# Autodesk Inventor assembly: TEST ASEMBLY
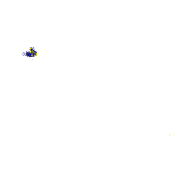
[picture p0: Inventor's stored thumbnail of the model, 180x180]
Saved by Autodesk Inventor 2019 (Build 230136000, 136)
## iProperties
Created: 2019-10-13
Part Number: TEST ASEMBLY
Document SubType Name: Assembly
Designer: Admin
Author: Admin
## Documents named in this file (21)
- C:\Users\Admin\Documents\TEST ASEMBLY.iam
- C:\Users\Admin\Documents\BASE FOR SYSTEM.ipt
- C:\Users\Admin\Documents\bolt for capping system.ipt
- C:\Users\Admin\Documents\bottom part of capping system.ipt
- C:\Users\Admin\Documents\nut for capping system.ipt
- C:\Users\Admin\Documents\without head nut for capping system.ipt
- C:\Users\Admin\Documents\cappingsystem 3rd part.ipt
- C:\Users\Admin\Documents\dc motor for capping system.ipt
- C:\Users\Admin\Documents\DC MOTOR NUT FOR CAPPING SYSTEM.ipt
- C:\Users\Admin\Documents\2 nd part of capping syStem.ipt
- C:\Users\Admin\Documents\two way connector for capping system.ipt
- C:\Users\Admin\Documents\CAPPER.ipt
- C:\Users\Admin\Documents\nut1.ipt
- C:\Users\Admin\Documents\STAND PLATE FOR STORSGE SYSTEM.ipt
- C:\Users\Admin\Documents\ir sensor.ipt
- C:\Users\Admin\Documents\top STAND PLATE FOR STORSGE SYSTEM.ipt
- C:\Users\Admin\Documents\Assembly3.iam
- C:\Users\Admin\Documents\ppe assembly.iam
- C:\Users\Admin\Documents\SA.ipt
- C:\Users\Admin\Documents\BOLT SMALL.ipt
- C:\Users\Admin\Documents\NUT FOR SERVO.ipt
## Components (63 placed, 20 different names)
1. BASE FOR SYSTEM:1 — Mate:1, Flush:1, Mate:2, Mate:3, Mate:4, Mate:5, Mate:6, Mate:7, Mate:8, Mate:9, Mate:10, Mate:13, Mate:14, Mate:65, Mate:66, Mate:68, Mate:69, Mate:70, Mate:72, Mate:77, Mate:142, Mate:143, Mate:144, Mate:145, Mate:146, Mate:149, Mate:150
2. bolt for capping system:1 — Mate:3, Mate:9, Mate:13, Mate:18, Mate:27, Mate:37, Mate:46, Mate:57
3. bolt for capping system:2 — Mate:4, Mate:7, Mate:16, Mate:28, Mate:38, Mate:47, Mate:54
4. bolt for capping system:3 — Mate:5, Mate:8, Mate:11, Mate:15, Mate:26, Mate:39, Mate:48, Mate:55
5. bolt for capping system:4 — Mate:6, Mate:10, Mate:12, Mate:17, Mate:25, Mate:36, Mate:49, Mate:56
6. bottom part of capping system:1 — Mate:11, Mate:12, Mate:14, Mate:19, Mate:20, Mate:21, Mate:22, Mate:23, Mate:24
7. nut for capping system:1 — Mate:15, Mate:21
8. nut for capping system:2 — Mate:17, Mate:19
9. nut for capping system:3 — Mate:16, Mate:20
10. nut for capping system:4 — Mate:18, Mate:22
11. without head nut for capping system:1 — Mate:23, Mate:24, Mate:29, Mate:30, Mate:112
12. cappingsystem 3rd part:1 — Mate:25, Mate:26, Mate:27, Mate:28, Mate:29, Mate:31, Mate:32, Mate:33, Mate:35
13. nut for capping system:5 — Mate:30, Mate:31
14. dc motor for capping system:1 — Mate:32, Mate:33, Mate:34, Mate:63
15. DC MOTOR NUT FOR CAPPING SYSTEM:1 — Mate:34, Mate:35, Mate:64
16. 2 nd part of capping syStem:1 — Mate:36, Mate:37, Mate:38, Mate:39, Mate:40, Mate:41, Mate:43, Mate:50, Mate:51, Mate:52, Mate:53, Mate:58, Mate:59, Mate:106, Mate:107
17. dc motor for capping system:2 — Mate:40, Mate:41, Mate:42, Mate:108
18. DC MOTOR NUT FOR CAPPING SYSTEM:2 — Mate:42, Mate:43, Mate:109
19. nut for capping system:6 — Mate:46, Mate:50
20. nut for capping system:7 — Mate:47, Mate:53
21. nut for capping system:8 — Mate:48, Mate:52
22. nut for capping system:9 — Mate:49, Mate:51
23. nut for capping system:10 — Mate:55, Mate:106
24. nut for capping system:11 — Mate:54, Mate:58
25. nut for capping system:12 — Mate:56, Mate:107
26. nut for capping system:13 — Mate:57, Mate:59
27. CAPPER:1 — Mate:63, Mate:64
28. nut1:1 — Mate:66, Mate:70, Mate:75, Mate:79, Mate:89, Mate:115, Mate:121
29. nut1:2 — Mate:65, Mate:69, Mate:76, Mate:81, Mate:87, Mate:113, Mate:122
30. nut1:3 — Mate:68, Mate:72, Mate:73, Mate:78, Mate:88, Mate:116, Mate:123
31. STAND PLATE FOR STORSGE SYSTEM:1 — Mate:73, Mate:75, Mate:76, Mate:77, Mate:82, Mate:83, Mate:84, Mate:85, Mate:141
32. nut for capping system:14 — Mate:78, Mate:82
33. nut for capping system:15 — Mate:79, Mate:84
34. nut for capping system:16 — Mate:85
35. nut for capping system:17 — Mate:81, Mate:83
36. nut for capping system:18 — Mate:119
37. nut for capping system:19 — Mate:87, Mate:120
38. nut for capping system:20 — Mate:89, Mate:117
39. nut for capping system:21 — Mate:88, Mate:118
40. ir sensor:1
41. two way connector for capping system:1 — Mate:108, Mate:109, Mate:110, Mate:111, Mate:112
42. two way connector for capping system:2 — Mate:110, Mate:111
43. top STAND PLATE FOR STORSGE SYSTEM:1 — Mate:113, Mate:115, Mate:116, Mate:117, Mate:118, Mate:119, Mate:120, Mate:125, Mate:126, Mate:127, Mate:128, Mate:129, Mate:130
44. nut for capping system:22 — Mate:121, Mate:128
45. nut for capping system:23 — Mate:122, Mate:127
46. nut for capping system:24 — Mate:126
47. nut for capping system:25 — Mate:123, Mate:125
48. Assembly3:1 [sub-assembly] — Mate:129, Mate:130
49. nut1:7 — Mate:141, Mate:142
50. SA:1 — Mate:144, Mate:146, Mate:147, Mate:152, Mate:154, Mate:157
51. SA:2 — Mate:143, Mate:145, Mate:148, Mate:151, Mate:153, Mate:158
52. nut for capping system:31 — Mate:147, Mate:149
53. nut for capping system:33 — Mate:148, Mate:150
54. nut for capping system:34
55. nut for capping system:35 — Mate:151, Mate:155
56. nut for capping system:36 — Mate:152, Mate:156
57. ppe assembly:1 [sub-assembly] — Mate:153, Mate:154, Mate:155, Mate:156, Mate:159, Mate:160, Mate:161, Mate:162
58. nut for capping system:37 — Mate:157, Mate:160
59. nut for capping system:38 — Mate:158, Mate:159
60. BOLT SMALL:3 — Mate:161, Mate:163
61. BOLT SMALL:4 — Mate:162, Mate:164
62. NUT FOR SERVO:1 — Mate:163
63. NUT FOR SERVO:2 — Mate:164
## Relationships (127: Mate 126, Flush 1)
- Mate:1: BASE FOR SYSTEM:1
- Flush:1: BASE FOR SYSTEM:1
- Mate:2: BASE FOR SYSTEM:1
- Mate:3: BASE FOR SYSTEM:1 ↔ bolt for capping system:1
- Mate:4: BASE FOR SYSTEM:1 ↔ bolt for capping system:2
- Mate:5: BASE FOR SYSTEM:1 ↔ bolt for capping system:3
- Mate:6: BASE FOR SYSTEM:1 ↔ bolt for capping system:4
- Mate:7: BASE FOR SYSTEM:1 ↔ bolt for capping system:2
- Mate:8: BASE FOR SYSTEM:1 ↔ bolt for capping system:3
- Mate:9: BASE FOR SYSTEM:1 ↔ bolt for capping system:1
- Mate:10: BASE FOR SYSTEM:1 ↔ bolt for capping system:4
- Mate:11: bolt for capping system:3 ↔ bottom part of capping system:1
- Mate:12: bolt for capping system:4 ↔ bottom part of capping system:1
- Mate:13: BASE FOR SYSTEM:1 ↔ bolt for capping system:1
- Mate:14: BASE FOR SYSTEM:1 ↔ bottom part of capping system:1
- Mate:15: bolt for capping system:3 ↔ nut for capping system:1
- Mate:16: bolt for capping system:2 ↔ nut for capping system:3
- Mate:17: bolt for capping system:4 ↔ nut for capping system:2
- Mate:18: bolt for capping system:1 ↔ nut for capping system:4
- Mate:19: bottom part of capping system:1 ↔ nut for capping system:2
- Mate:20: bottom part of capping system:1 ↔ nut for capping system:3
- Mate:21: bottom part of capping system:1 ↔ nut for capping system:1
- Mate:22: bottom part of capping system:1 ↔ nut for capping system:4
- Mate:23: bottom part of capping system:1 ↔ without head nut for capping system:1
- Mate:24: bottom part of capping system:1 ↔ without head nut for capping system:1
- Mate:25: bolt for capping system:4 ↔ cappingsystem 3rd part:1
- Mate:26: bolt for capping system:3 ↔ cappingsystem 3rd part:1
- Mate:27: bolt for capping system:1 ↔ cappingsystem 3rd part:1
- Mate:28: bolt for capping system:2 ↔ cappingsystem 3rd part:1
- Mate:29: without head nut for capping system:1 ↔ cappingsystem 3rd part:1
- Mate:30: without head nut for capping system:1 ↔ nut for capping system:5
- Mate:31: cappingsystem 3rd part:1 ↔ nut for capping system:5
- Mate:32: cappingsystem 3rd part:1 ↔ dc motor for capping system:1
- Mate:33: cappingsystem 3rd part:1 ↔ dc motor for capping system:1
- Mate:34: dc motor for capping system:1 ↔ DC MOTOR NUT FOR CAPPING SYSTEM:1
- Mate:35: cappingsystem 3rd part:1 ↔ DC MOTOR NUT FOR CAPPING SYSTEM:1
- Mate:36: bolt for capping system:4 ↔ 2 nd part of capping syStem:1
- Mate:37: bolt for capping system:1 ↔ 2 nd part of capping syStem:1
- Mate:38: bolt for capping system:2 ↔ 2 nd part of capping syStem:1
- Mate:39: bolt for capping system:3 ↔ 2 nd part of capping syStem:1
- Mate:40: 2 nd part of capping syStem:1 ↔ dc motor for capping system:2
- Mate:41: 2 nd part of capping syStem:1 ↔ dc motor for capping system:2
- Mate:42: dc motor for capping system:2 ↔ DC MOTOR NUT FOR CAPPING SYSTEM:2
- Mate:43: 2 nd part of capping syStem:1 ↔ DC MOTOR NUT FOR CAPPING SYSTEM:2
- Mate:46: bolt for capping system:1 ↔ nut for capping system:6
- Mate:47: bolt for capping system:2 ↔ nut for capping system:7
- Mate:48: bolt for capping system:3 ↔ nut for capping system:8
- Mate:49: bolt for capping system:4 ↔ nut for capping system:9
- Mate:50: 2 nd part of capping syStem:1 ↔ nut for capping system:6
- Mate:51: 2 nd part of capping syStem:1 ↔ nut for capping system:9
- Mate:52: 2 nd part of capping syStem:1 ↔ nut for capping system:8
- Mate:53: 2 nd part of capping syStem:1 ↔ nut for capping system:7
- Mate:54: bolt for capping system:2 ↔ nut for capping system:11
- Mate:55: bolt for capping system:3 ↔ nut for capping system:10
- Mate:56: bolt for capping system:4 ↔ nut for capping system:12
- Mate:57: bolt for capping system:1 ↔ nut for capping system:13
- Mate:58: 2 nd part of capping syStem:1 ↔ nut for capping system:11
- Mate:59: 2 nd part of capping syStem:1 ↔ nut for capping system:13
- Mate:63: dc motor for capping system:1 ↔ CAPPER:1
- Mate:64: DC MOTOR NUT FOR CAPPING SYSTEM:1 ↔ CAPPER:1
- Mate:65: BASE FOR SYSTEM:1 ↔ nut1:2
- Mate:66: BASE FOR SYSTEM:1 ↔ nut1:1
- Mate:68: BASE FOR SYSTEM:1 ↔ nut1:3
- Mate:69: BASE FOR SYSTEM:1 ↔ nut1:2
- Mate:70: BASE FOR SYSTEM:1 ↔ nut1:1
- Mate:72: BASE FOR SYSTEM:1 ↔ nut1:3
- Mate:73: nut1:3 ↔ STAND PLATE FOR STORSGE SYSTEM:1
- Mate:75: nut1:1 ↔ STAND PLATE FOR STORSGE SYSTEM:1
- Mate:76: nut1:2 ↔ STAND PLATE FOR STORSGE SYSTEM:1
- Mate:77: BASE FOR SYSTEM:1 ↔ STAND PLATE FOR STORSGE SYSTEM:1
- Mate:78: nut1:3 ↔ nut for capping system:14
- Mate:79: nut1:1 ↔ nut for capping system:15
- Mate:81: nut1:2 ↔ nut for capping system:17
- Mate:82: STAND PLATE FOR STORSGE SYSTEM:1 ↔ nut for capping system:14
- Mate:83: STAND PLATE FOR STORSGE SYSTEM:1 ↔ nut for capping system:17
- Mate:84: STAND PLATE FOR STORSGE SYSTEM:1 ↔ nut for capping system:15
- Mate:85: STAND PLATE FOR STORSGE SYSTEM:1 ↔ nut for capping system:16
- Mate:87: nut1:2 ↔ nut for capping system:19
- Mate:88: nut1:3 ↔ nut for capping system:21
- Mate:89: nut1:1 ↔ nut for capping system:20
- Mate:106: 2 nd part of capping syStem:1 ↔ nut for capping system:10
- Mate:107: 2 nd part of capping syStem:1 ↔ nut for capping system:12
- Mate:108: dc motor for capping system:2 ↔ two way connector for capping system:1
- Mate:109: DC MOTOR NUT FOR CAPPING SYSTEM:2 ↔ two way connector for capping system:1
- Mate:110: two way connector for capping system:1 ↔ two way connector for capping system:2
- Mate:111: two way connector for capping system:1 ↔ two way connector for capping system:2
- Mate:112: without head nut for capping system:1 ↔ two way connector for capping system:1
- Mate:113: nut1:2 ↔ top STAND PLATE FOR STORSGE SYSTEM:1
- Mate:115: nut1:1 ↔ top STAND PLATE FOR STORSGE SYSTEM:1
- Mate:116: nut1:3 ↔ top STAND PLATE FOR STORSGE SYSTEM:1
- Mate:117: nut for capping system:20 ↔ top STAND PLATE FOR STORSGE SYSTEM:1
- Mate:118: nut for capping system:21 ↔ top STAND PLATE FOR STORSGE SYSTEM:1
- Mate:119: nut for capping system:18 ↔ top STAND PLATE FOR STORSGE SYSTEM:1
- Mate:120: nut for capping system:19 ↔ top STAND PLATE FOR STORSGE SYSTEM:1
- Mate:121: nut1:1 ↔ nut for capping system:22
- Mate:122: nut1:2 ↔ nut for capping system:23
- Mate:123: nut1:3 ↔ nut for capping system:25
- Mate:125: top STAND PLATE FOR STORSGE SYSTEM:1 ↔ nut for capping system:25
- Mate:126: top STAND PLATE FOR STORSGE SYSTEM:1 ↔ nut for capping system:24
- Mate:127: top STAND PLATE FOR STORSGE SYSTEM:1 ↔ nut for capping system:23
- Mate:128: top STAND PLATE FOR STORSGE SYSTEM:1 ↔ nut for capping system:22
- Mate:129: top STAND PLATE FOR STORSGE SYSTEM:1 ↔ Assembly3:1
- Mate:130: top STAND PLATE FOR STORSGE SYSTEM:1 ↔ Assembly3:1
- Mate:141: STAND PLATE FOR STORSGE SYSTEM:1 ↔ nut1:7
- Mate:142: BASE FOR SYSTEM:1 ↔ nut1:7
- Mate:143: BASE FOR SYSTEM:1 ↔ SA:2
- Mate:144: BASE FOR SYSTEM:1 ↔ SA:1
- Mate:145: BASE FOR SYSTEM:1 ↔ SA:2
- Mate:146: BASE FOR SYSTEM:1 ↔ SA:1
- Mate:147: SA:1 ↔ nut for capping system:31
- Mate:148: SA:2 ↔ nut for capping system:33
- Mate:149: BASE FOR SYSTEM:1 ↔ nut for capping system:31
- Mate:150: BASE FOR SYSTEM:1 ↔ nut for capping system:33
- Mate:151: SA:2 ↔ nut for capping system:35
- Mate:152: SA:1 ↔ nut for capping system:36
- Mate:153: SA:2 ↔ ppe assembly:1
- Mate:154: SA:1 ↔ ppe assembly:1
- Mate:155: nut for capping system:35 ↔ ppe assembly:1
- Mate:156: nut for capping system:36 ↔ ppe assembly:1
- Mate:157: SA:1 ↔ nut for capping system:37
- Mate:158: SA:2 ↔ nut for capping system:38
- Mate:159: ppe assembly:1 ↔ nut for capping system:38
- Mate:160: ppe assembly:1 ↔ nut for capping system:37
- Mate:161: ppe assembly:1 ↔ BOLT SMALL:3
- Mate:162: ppe assembly:1 ↔ BOLT SMALL:4
- Mate:163: BOLT SMALL:3 ↔ NUT FOR SERVO:1
- Mate:164: BOLT SMALL:4 ↔ NUT FOR SERVO:2
